# Autodesk Inventor assembly: Drive2
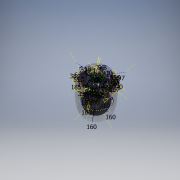
[picture p0: Inventor's stored thumbnail of the model, 180x180]
Saved by Autodesk Inventor 2018.3 (Build 223284000, 284)
## iProperties
Created: 2018-06-30
Part Number: Drive2
Material: Generisch
Document SubType Name: Assembly
Designer: JochenAlt
Author: JochenAlt
## Documents named in this file (4)
- D:\Projects\FlowerPot\CAD\Drive.iam
- D:\Projects\FlowerPot\CAD\Sphere.ipt
- D:\Projects\FlowerPot\CAD\Form.iam
- D:\Projects\FlowerPot\CAD\DriveChain.iam
## Components (5 placed, 3 different names)
1. Sphere:1 — Passend:38, Tangential:1
2. Form:1 [sub-assembly] — Passend:60, Passend:61
3. DriveChain:1 [sub-assembly] — Passend:51, Passend:55, Passend:57, Passend:58, Passend:61
4. DriveChain:2 [sub-assembly] — Passend:51, Passend:55, Passend:56, Passend:60, Tangential:1
5. DriveChain:3 [sub-assembly] — Passend:56, Passend:57
## Relationships (9: Mate 8, Tangent 1)
- Passend:38 [Mate]: Sphere:1
- Passend:51 [Mate]: DriveChain:1 ↔ DriveChain:2
- Passend:55 [Mate]: DriveChain:1 ↔ DriveChain:2
- Passend:56 [Mate]: DriveChain:2 ↔ DriveChain:3
- Passend:57 [Mate]: DriveChain:1 ↔ DriveChain:3
- Passend:58 [Mate]: DriveChain:1
- Passend:60 [Mate]: Form:1 ↔ DriveChain:2
- Tangential:1: Sphere:1 ↔ DriveChain:2
- Passend:61 [Mate]: Form:1 ↔ DriveChain:1
